# Autodesk Inventor assembly: assembly_CIntake
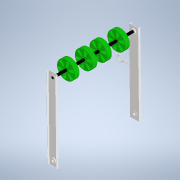
[picture p0: Inventor's stored thumbnail of the model, 180x180]
Saved by Autodesk Inventor 2021.1 (Build 251245000, 245)
## iProperties
Created: 2021-02-27
Part Number: assembly_CIntake
Document SubType Name: Assembly
Designer: JavDiazV
Author: JavDiazV
## Documents named in this file (6)
- C:\Users\Spade\OneDrive\Documents\t3-cad\CAD\Javier's CAD\assembly_CIntake.iam
- C:\Users\Spade\OneDrive\Documents\t3-cad\CAD\Javier's CAD\VerseFrameCChannel 18in.ipt
- C:\Users\Spade\OneDrive\Documents\t3-cad\CAD\Javier's CAD\part_ Ball Bearing for Thundershaft.ipt
- C:\Users\Spade\OneDrive\Documents\t3-cad\CAD\Javier's CAD\part_18 in. Thundershaft.ipt
- C:\Users\Spade\OneDrive\Documents\t3-cad\CAD\Javier's CAD\JHook.ipt
- C:\Users\Spade\OneDrive\Documents\t3-cad\CAD\Javier's CAD\part_4 in. Compliance Wheel.ipt
## Components (12 placed, 5 different names)
1. VerseFrameCChannel 18in:1 — Insert:2, Flush:1, Flush:2, Insert:9
2. VerseFrameCChannel 18in:3 — Insert:4, Flush:1, Flush:2, Insert:8, Insert:10
3. part_ Ball Bearing for Thundershaft:1 — Insert:5, Insert:8
4. part_ Ball Bearing for Thundershaft:2 — Insert:4
5. part_ Ball Bearing for Thundershaft:3 — Insert:6, Insert:9
6. part_ Ball Bearing for Thundershaft:4 — Insert:2
7. part_18 in. Thundershaft:1 — Insert:5, Insert:6, Insert:11, Insert:12, Insert:13, Insert:14
8. JHook:1 — Insert:10
9. part_4 in. Compliance Wheel:1 — Insert:11
10. part_4 in. Compliance Wheel:2 — Insert:12
11. part_4 in. Compliance Wheel:3 — Insert:13
12. part_4 in. Compliance Wheel:4 — Insert:14
## Relationships (13: Insert 11, Flush 2)
- Insert:2: VerseFrameCChannel 18in:1 ↔ part_ Ball Bearing for Thundershaft:4
- Insert:4: VerseFrameCChannel 18in:3 ↔ part_ Ball Bearing for Thundershaft:2
- Insert:5: part_ Ball Bearing for Thundershaft:1 ↔ part_18 in. Thundershaft:1
- Insert:6: part_ Ball Bearing for Thundershaft:3 ↔ part_18 in. Thundershaft:1
- Flush:1: VerseFrameCChannel 18in:1 ↔ VerseFrameCChannel 18in:3
- Flush:2: VerseFrameCChannel 18in:1 ↔ VerseFrameCChannel 18in:3
- Insert:8: VerseFrameCChannel 18in:3 ↔ part_ Ball Bearing for Thundershaft:1
- Insert:9: VerseFrameCChannel 18in:1 ↔ part_ Ball Bearing for Thundershaft:3
- Insert:10: VerseFrameCChannel 18in:3 ↔ JHook:1
- Insert:11 (-101.6 mm): part_18 in. Thundershaft:1 ↔ part_4 in. Compliance Wheel:1
- Insert:12 (-203.2 mm): part_18 in. Thundershaft:1 ↔ part_4 in. Compliance Wheel:2
- Insert:13 (-203.2 mm): part_18 in. Thundershaft:1 ↔ part_4 in. Compliance Wheel:3
- Insert:14 (-101.6 mm): part_18 in. Thundershaft:1 ↔ part_4 in. Compliance Wheel:4
